# Autodesk Inventor assembly: manipulator
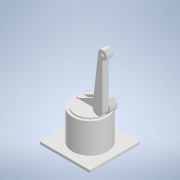
[picture p0: Inventor's stored thumbnail of the model, 180x180]
Saved by Autodesk Inventor 2022.2 (Build 262287010, 287A)
## iProperties
Created: 2022-04-10
Part Number: manipulator
Document SubType Name: Assembly
Designer: stasi
Author: stasi
## Documents named in this file (4)
- D:\stuff\P G\sem6\KPMiR\proj\KPMiR_RRR_BGD\manipulator.iam
- D:\stuff\P G\sem6\KPMiR\proj\KPMiR_RRR_BGD\C0.ipt
- D:\stuff\P G\sem6\KPMiR\proj\KPMiR_RRR_BGD\C1.ipt
- C:\Users\stasi\Documents\C2.ipt
## Components (3 placed, 3 different names)
1. C0:1 — Flush:1, Flush:3
2. C1:1 — Flush:1, Flush:3, Flush:4, Flush:5
3. C2:1 — Flush:4, Flush:5
## Relationships (4: Flush 4)
- Flush:1: C0:1 ↔ C1:1
- Flush:3: C0:1 ↔ C1:1
- Flush:4: C1:1 ↔ C2:1
- Flush:5: C1:1 ↔ C2:1
